# Autodesk Inventor assembly: MecanumWheel2.0
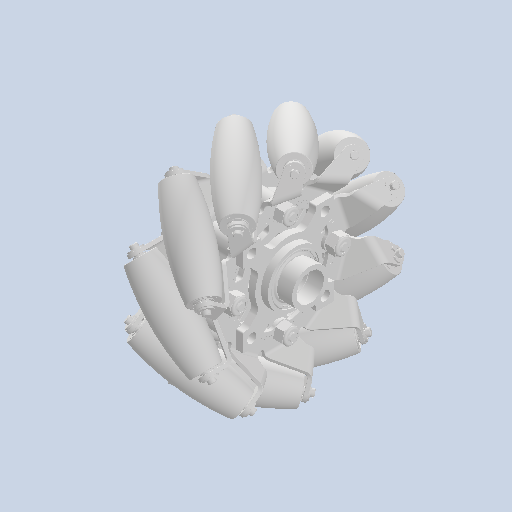
[picture p0: Inventor's stored thumbnail of the model, 512x512]
Saved by Autodesk Inventor 2023 (Build 270158000, 158)
## iProperties
Created: 2022-09-23
Part Number: MecanumWheel2.0
Document SubType Name: Assembly
Designer: deli
Author: deli
## Documents named in this file (6)
- C:\Users\deli\OneDrive - Eastside Preparatory School\FTC\8103-power-play\CAD\MecanumWheel2.0.iam
- C:\Users\deli\OneDrive - Eastside Preparatory School\FTC\8103-power-play\CAD\FTC-parts\goBILDA\3213-3606-0002\3606-0000-0096 assembly.ipt
- C:\Users\deli\OneDrive - Eastside Preparatory School\FTC\8103-power-play\CAD\FTC-parts\goBILDA\1603-0032-0012 assembly.ipt
- C:\Users\deli\OneDrive - Eastside Preparatory School\FTC\8103-power-play\CAD\wheelBearingInside2.0.ipt
- C:\Users\deli\OneDrive - Eastside Preparatory School\FTC\8103-power-play\CAD\20.5mmSpacer.ipt
- C:\Users\deli\OneDrive - Eastside Preparatory School\FTC\8103-power-play\CAD\6.5mmSpacer.ipt
## Components (6 placed, 5 different names)
1. 3606-0000-0096 assembly:1 — Mate:1, Mate:2, Mate:3, Mate:4, Mate:5, Mate:6
2. 1603-0032-0012 assembly:1 — Mate:1, Mate:2, Mate:3, Mate:13, Mate:14
3. 1603-0032-0012 assembly:2 — Mate:4, Mate:5, Mate:6, Mate:7, Mate:8, Mate:9, Mate:12
4. wheelBearingInside2.0:1 — Mate:7, Mate:8, Mate:9
5. 20.5mmSpacer:1 — Mate:12
6. 6.5mmSpacer:1 — Mate:13, Mate:14
## Relationships (12: Mate 12)
- Mate:1: 3606-0000-0096 assembly:1 ↔ 1603-0032-0012 assembly:1
- Mate:2: 3606-0000-0096 assembly:1 ↔ 1603-0032-0012 assembly:1
- Mate:3: 3606-0000-0096 assembly:1 ↔ 1603-0032-0012 assembly:1
- Mate:4: 3606-0000-0096 assembly:1 ↔ 1603-0032-0012 assembly:2
- Mate:5: 3606-0000-0096 assembly:1 ↔ 1603-0032-0012 assembly:2
- Mate:6: 3606-0000-0096 assembly:1 ↔ 1603-0032-0012 assembly:2
- Mate:7: 1603-0032-0012 assembly:2 ↔ wheelBearingInside2.0:1
- Mate:8: 1603-0032-0012 assembly:2 ↔ wheelBearingInside2.0:1
- Mate:9: 1603-0032-0012 assembly:2 ↔ wheelBearingInside2.0:1
- Mate:12: 1603-0032-0012 assembly:2 ↔ 20.5mmSpacer:1
- Mate:13: 1603-0032-0012 assembly:1 ↔ 6.5mmSpacer:1
- Mate:14: 1603-0032-0012 assembly:1 ↔ 6.5mmSpacer:1
